# Autodesk Inventor assembly: Chasis inferior _1_
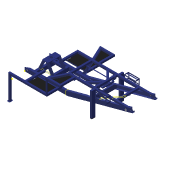
[picture p0: Inventor's stored thumbnail of the model, 180x180]
Saved by Autodesk Inventor 2019 (Build 230136000, 136)
## iProperties
Created: 2020-02-06
Part Number: Chasis inferior _1_
Document SubType Name: Assembly
Designer: Juan Carlos Botero
Author: Juan Carlos Botero
## Documents named in this file (52)
- D:\Drives\OneDrive\Carlos_2\02 TRABAJOS\MULTIPLO\Conveyor\ENSAMBLE\Chasis inferior _1_.iam
- D:\Drives\OneDrive\Carlos_2\02 TRABAJOS\MULTIPLO\Conveyor\ENSAMBLE\Refuerzo diagonal tiro.ipt
- D:\Drives\OneDrive\Carlos_2\02 TRABAJOS\MULTIPLO\Conveyor\ENSAMBLE\Lamina escalon 2.ipt
- D:\Drives\OneDrive\Carlos_2\02 TRABAJOS\MULTIPLO\Conveyor\ENSAMBLE\Lamina sujeción bateria 2.ipt
- D:\Drives\OneDrive\Carlos_2\02 TRABAJOS\MULTIPLO\Conveyor\ENSAMBLE\Refuerzo perfil en C.ipt
- D:\Drives\OneDrive\Carlos_2\02 TRABAJOS\MULTIPLO\Conveyor\ENSAMBLE\Tapa perfil 100x50.ipt
- D:\Drives\OneDrive\Carlos_2\02 TRABAJOS\MULTIPLO\Conveyor\ENSAMBLE\Angulo soporte batería 1.ipt
- D:\Drives\OneDrive\Carlos_2\02 TRABAJOS\MULTIPLO\Conveyor\ENSAMBLE\Perfil 1 en C derecho 2.ipt
- D:\Drives\OneDrive\Carlos_2\02 TRABAJOS\MULTIPLO\Conveyor\ENSAMBLE\Unión vigas chasis.ipt
- D:\Drives\OneDrive\Carlos_2\02 TRABAJOS\MULTIPLO\Conveyor\ENSAMBLE\Caucho tope banda.ipt
- D:\Drives\OneDrive\Carlos_2\02 TRABAJOS\MULTIPLO\Conveyor\ENSAMBLE\Refuerzo diagonal chasis inferior.ipt
- D:\Drives\OneDrive\Carlos_2\02 TRABAJOS\MULTIPLO\Conveyor\ENSAMBLE\Perfil escalón 6.ipt
- D:\Drives\OneDrive\Carlos_2\02 TRABAJOS\MULTIPLO\Conveyor\ENSAMBLE\Perfil escalón 3.ipt
- D:\Drives\OneDrive\Carlos_2\02 TRABAJOS\MULTIPLO\Conveyor\ENSAMBLE\Espaciador de nylon.ipt
- D:\Drives\OneDrive\Carlos_2\02 TRABAJOS\MULTIPLO\Conveyor\ENSAMBLE\Refuerzo chasis.ipt
- D:\Drives\OneDrive\Carlos_2\02 TRABAJOS\MULTIPLO\Conveyor\ENSAMBLE\Perfil escalón 4.ipt
- D:\Drives\OneDrive\Carlos_2\02 TRABAJOS\MULTIPLO\Conveyor\ENSAMBLE\Tope banda.ipt
- D:\Drives\OneDrive\Carlos_2\02 TRABAJOS\MULTIPLO\Conveyor\ENSAMBLE\Buje.ipt
- D:\Drives\OneDrive\Carlos_2\02 TRABAJOS\MULTIPLO\Conveyor\ENSAMBLE\Lamina indexacion eje trasero.ipt
- D:\Drives\OneDrive\Carlos_2\02 TRABAJOS\MULTIPLO\Conveyor\ENSAMBLE\Refuerzo horizontal tiro.ipt
- D:\Drives\OneDrive\Carlos_2\02 TRABAJOS\MULTIPLO\Conveyor\ENSAMBLE\Angulo escalón 1.ipt
- D:\Drives\OneDrive\Carlos_2\02 TRABAJOS\MULTIPLO\Conveyor\ENSAMBLE\Base chasis inferior izquierdo.ipt
- D:\Drives\OneDrive\Carlos_2\02 TRABAJOS\MULTIPLO\Conveyor\ENSAMBLE\Refuerzo diagonal estructura tiro.ipt
- D:\Drives\OneDrive\Carlos_2\02 TRABAJOS\MULTIPLO\Conveyor\ENSAMBLE\Perfil 1 en C izquierdo 2.ipt
- D:\Drives\OneDrive\Carlos_2\02 TRABAJOS\MULTIPLO\Conveyor\ENSAMBLE\Lamina escalon 1.ipt
- D:\Drives\OneDrive\Carlos_2\02 TRABAJOS\MULTIPLO\Conveyor\ENSAMBLE\Lamina pivote actuador lineal pequeño.ipt
- D:\Drives\OneDrive\Carlos_2\02 TRABAJOS\MULTIPLO\Conveyor\ENSAMBLE\Perfil 1 en C izquierdo 1.ipt
- D:\Drives\OneDrive\Carlos_2\02 TRABAJOS\MULTIPLO\Conveyor\ENSAMBLE\Perfil 1 en C derecho 1.ipt
- D:\Drives\OneDrive\Carlos_2\02 TRABAJOS\MULTIPLO\Conveyor\ENSAMBLE\Lamina baliza.ipt
- D:\Drives\OneDrive\Carlos_2\02 TRABAJOS\MULTIPLO\Conveyor\ENSAMBLE\Perfil escalón 2.ipt
- D:\Drives\OneDrive\Carlos_2\02 TRABAJOS\MULTIPLO\Conveyor\ENSAMBLE\Perfil escalón 5.ipt
- D:\Drives\OneDrive\Carlos_2\02 TRABAJOS\MULTIPLO\Conveyor\ENSAMBLE\Espaciador pivote 1.ipt
- D:\Drives\OneDrive\Carlos_2\02 TRABAJOS\MULTIPLO\Conveyor\ENSAMBLE\Platina inferior actuador lineal.ipt
- D:\Drives\OneDrive\Carlos_2\02 TRABAJOS\MULTIPLO\Conveyor\ENSAMBLE\Angulo escalón 3.ipt
- D:\Drives\OneDrive\Carlos_2\02 TRABAJOS\MULTIPLO\Conveyor\ENSAMBLE\Refuerzo diagonal.ipt
- D:\Drives\OneDrive\Carlos_2\02 TRABAJOS\MULTIPLO\Conveyor\ENSAMBLE\Perfil escalón 1.ipt
- D:\Drives\OneDrive\Carlos_2\02 TRABAJOS\MULTIPLO\Conveyor\ENSAMBLE\Pie amigo lamina quinta rueda.ipt
- D:\Drives\OneDrive\Carlos_2\02 TRABAJOS\MULTIPLO\Conveyor\ENSAMBLE\Perfil 2 en C derecho.ipt
- D:\Drives\OneDrive\Carlos_2\02 TRABAJOS\MULTIPLO\Conveyor\ENSAMBLE\Espaciador pivote 2.ipt
- D:\Drives\OneDrive\Carlos_2\02 TRABAJOS\MULTIPLO\Conveyor\ENSAMBLE\Perfil 2 en C izquierdo.ipt
- D:\Drives\OneDrive\Carlos_2\02 TRABAJOS\MULTIPLO\Conveyor\ENSAMBLE\Lamina pivote quinta rueda.ipt
- D:\Drives\OneDrive\Carlos_2\02 TRABAJOS\MULTIPLO\Conveyor\ENSAMBLE\Angulo soporte batería 3.ipt
- D:\Drives\OneDrive\Carlos_2\02 TRABAJOS\MULTIPLO\Conveyor\ENSAMBLE\Angulo soporte batería 2.ipt
- D:\Drives\OneDrive\Carlos_2\02 TRABAJOS\MULTIPLO\Conveyor\ENSAMBLE\Unión base chasis inferior.ipt
- D:\Drives\OneDrive\Carlos_2\02 TRABAJOS\MULTIPLO\Conveyor\ENSAMBLE\Soporte baliza.ipt
- D:\Drives\OneDrive\Carlos_2\02 TRABAJOS\MULTIPLO\Conveyor\ENSAMBLE\Base chasis inferior derecho.ipt
- D:\Drives\OneDrive\Carlos_2\02 TRABAJOS\MULTIPLO\Conveyor\ENSAMBLE\Refuerzo intermedio.ipt
- D:\Drives\OneDrive\Carlos_2\02 TRABAJOS\MULTIPLO\Conveyor\ENSAMBLE\Ensamble cuñas y soporte _1_.iam
- D:\Drives\OneDrive\Carlos_2\02 TRABAJOS\MULTIPLO\Conveyor\ENSAMBLE\Ensamble cuñas y soporte _1__1.iam
- D:\Drives\OneDrive\Carlos_2\02 TRABAJOS\MULTIPLO\Conveyor\ENSAMBLE\sketch.ipt
- D:\Drives\OneDrive\Carlos_2\02 TRABAJOS\MULTIPLO\Conveyor\ENSAMBLE\Barra nuevo pivote.ipt
- D:\Drives\OneDrive\Carlos_2\02 TRABAJOS\MULTIPLO\Conveyor\ENSAMBLE\Perfil refuerzo.ipt
## Components (98 placed, 50 different names)
1. Refuerzo diagonal tiro:1 — Mate:6
2. Lamina escalon 2:1
3. Lamina sujeción bateria 2:1
4. Lamina escalon 2:2
5. Refuerzo perfil en C:1 — Flush:10
6. Tapa perfil 100x50:1
7. Angulo soporte batería 1:1
8. Perfil 1 en C derecho 2:1 — Flush:8, Flush:13
9. Unión vigas chasis:1
10. Caucho tope banda:1
11. Refuerzo diagonal chasis inferior:1
12. Perfil escalón 6:1
13. Perfil escalón 3:1
14. Refuerzo perfil en C:2 — Flush:12
15. Espaciador de nylon:1
16. Refuerzo chasis:1
17. Perfil escalón 4:1
18. Tope banda:1
19. Buje:1
20. Perfil escalón 3:2
21. Lamina indexacion eje trasero:1
22. Refuerzo horizontal tiro:1
23. Angulo escalón 1:1
24. Base chasis inferior izquierdo:1
25. Perfil escalón 3:3
26. Lamina indexacion eje trasero:2
27. Refuerzo horizontal tiro:2 — Flush:6, Flush:7
28. Caucho tope banda:2
29. Refuerzo diagonal estructura tiro:1 — Mate:3, Mate:5
30. Refuerzo diagonal tiro:2 — Flush:6, Mate:8
31. Perfil 1 en C izquierdo 2:1 — Flush:2, Flush:11
32. Tapa perfil 100x50:2
33. Refuerzo diagonal chasis inferior:2
34. Lamina escalon 1:1
35. Lamina pivote actuador lineal pequeño:1
36. Perfil 1 en C izquierdo 1:1
37. Perfil 1 en C derecho 1:1
38. Lamina baliza:1
39. Perfil escalón 2:1
40. Perfil escalón 5:1
41. Perfil escalón 5:2
42. Lamina pivote actuador lineal pequeño:2
43. Espaciador pivote 1:1
44. Refuerzo chasis:2
45. Unión vigas chasis:2
46. Perfil escalón 3:4
47. Platina inferior actuador lineal:1
48. Espaciador pivote 1:2
49. Buje:3
50. Perfil escalón 3:5
51. Angulo escalón 3:1
52. Refuerzo diagonal:1
53. Espaciador de nylon:3
54. Refuerzo diagonal estructura tiro:2 — Flush:7
55. Perfil escalón 1:1 — Mate:1
56. Pie amigo lamina quinta rueda:1
57. Perfil 2 en C derecho:1
58. Tapa perfil 100x50:3
59. Perfil escalón 4:2
60. Perfil 2 en C izquierdo:1
61. Refuerzo diagonal:2
62. Angulo escalón 3:2
63. Pie amigo lamina quinta rueda:2
64. Platina inferior actuador lineal:2
65. Tope banda:2
66. Refuerzo chasis:3
67. Tapa perfil 100x50:4
68. Platina inferior actuador lineal:3
69. Pie amigo lamina quinta rueda:3
70. Lamina pivote quinta rueda:1
71. Angulo soporte batería 3:1
72. Angulo soporte batería 2:1
73. Perfil escalón 2:2
74. Angulo soporte batería 3:2
75. Pie amigo lamina quinta rueda:4
76. Unión base chasis inferior:1
77. Perfil escalón 6:2
78. Soporte baliza:1
79. Lamina escalon 1:2
80. Base chasis inferior derecho:1
81. Angulo escalón 1:2
82. Refuerzo intermedio:1
83. Perfil escalón 1:2 — Mate:2
84. Refuerzo intermedio:2
85. Platina inferior actuador lineal:4
86. Ensamble cuñas y soporte <1>:1 [sub-assembly]
87. Ensamble cuñas y soporte <1>:2 [sub-assembly]
88. sketch:1 — Flush:1
89. Barra nuevo pivote:1 — Flush:2, Mate:1, Flush:5, Flush:9, Flush:10, Flush:11
90. Barra nuevo pivote:2 — Mate:2, Flush:8, Flush:9, Mate:4, Mate:7, Flush:12, Flush:13
91. Perfil refuerzo:1 — Mate:3, Mate:4, Mate:5
92. Perfil refuerzo:2 — Mate:6, Mate:7, Mate:8
93. Buje:2
94. Espaciador de nylon:2
95. Espaciador pivote 2:1
96. Espaciador de nylon:4
97. Espaciador pivote 2:2
98. Buje:4
## Relationships (19: Flush 11, Mate 8)
- Flush:1: sketch:1
- Flush:2: Perfil 1 en C izquierdo 2:1 ↔ Barra nuevo pivote:1
- Mate:1: Perfil escalón 1:1 ↔ Barra nuevo pivote:1
- Flush:5: Barra nuevo pivote:1
- Flush:6: Refuerzo horizontal tiro:2 ↔ Refuerzo diagonal tiro:2
- Flush:7: Refuerzo horizontal tiro:2 ↔ Refuerzo diagonal estructura tiro:2
- Mate:2: Perfil escalón 1:2 ↔ Barra nuevo pivote:2
- Flush:8 (12.013 mm): Perfil 1 en C derecho 2:1 ↔ Barra nuevo pivote:2
- Flush:9: Barra nuevo pivote:1 ↔ Barra nuevo pivote:2
- Mate:3: Refuerzo diagonal estructura tiro:1 ↔ Perfil refuerzo:1
- Mate:4: Barra nuevo pivote:2 ↔ Perfil refuerzo:1
- Mate:5: Refuerzo diagonal estructura tiro:1 ↔ Perfil refuerzo:1
- Mate:6: Refuerzo diagonal tiro:1 ↔ Perfil refuerzo:2
- Mate:7: Barra nuevo pivote:2 ↔ Perfil refuerzo:2
- Mate:8: Refuerzo diagonal tiro:2 ↔ Perfil refuerzo:2
- Flush:10: Refuerzo perfil en C:1 ↔ Barra nuevo pivote:1
- Flush:11: Perfil 1 en C izquierdo 2:1 ↔ Barra nuevo pivote:1
- Flush:12: Refuerzo perfil en C:2 ↔ Barra nuevo pivote:2
- Flush:13: Perfil 1 en C derecho 2:1 ↔ Barra nuevo pivote:2
